# Autodesk Inventor assembly: testSupportPoket
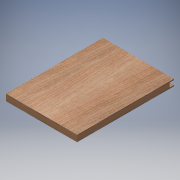
[picture p0: Inventor's stored thumbnail of the model, 180x180]
Saved by Autodesk Inventor 2019 (Build 230136000, 136)
## iProperties
Created: 2019-02-01
Part Number: testSupportPoket
Document SubType Name: Assembly
Designer: gaincarlo
Author: gaincarlo
## Documents named in this file (4)
- D:\Giancarlo Bacchio\Documenti\00 - Progetti\30-Inventor\flower vase\testSupportPoket.iam
- D:\Giancarlo Bacchio\Documenti\00 - Progetti\30-Inventor\flower vase\testSupport_parts\testBasePlate.ipt
- D:\Giancarlo Bacchio\Documenti\00 - Progetti\30-Inventor\flower vase\testSupport_parts\testsideLong.ipt
- D:\Giancarlo Bacchio\Documenti\00 - Progetti\30-Inventor\flower vase\testSupport_parts\testsideShort.ipt
## Components (5 placed, 3 different names)
1. testBasePlate:1 — Flush:1, Mate:1, Flush:2, Mate:2, Flush:3, Mate:7
2. testsideLong:1 — Flush:2, Mate:2, Mate:3, Flush:8
3. testsideLong:2 — Mate:6, Flush:6, Mate:7, Mate:8
4. testsideShort:1 — Flush:1, Mate:1, Mate:3, Flush:3, Mate:6, Flush:6, Flush:7
5. testBasePlate:2 — Flush:7, Mate:8, Flush:8
## Relationships (12: Flush 6, Mate 6)
- Flush:1: testBasePlate:1 ↔ testsideShort:1
- Mate:1: testBasePlate:1 ↔ testsideShort:1
- Flush:2: testBasePlate:1 ↔ testsideLong:1
- Mate:2: testBasePlate:1 ↔ testsideLong:1
- Mate:3: testsideLong:1 ↔ testsideShort:1
- Flush:3: testBasePlate:1 ↔ testsideShort:1
- Mate:6: testsideLong:2 ↔ testsideShort:1
- Flush:6: testsideLong:2 ↔ testsideShort:1
- Mate:7: testBasePlate:1 ↔ testsideLong:2
- Flush:7: testsideShort:1 ↔ testBasePlate:2
- Mate:8: testsideLong:2 ↔ testBasePlate:2
- Flush:8: testsideLong:1 ↔ testBasePlate:2
